# Autodesk Inventor assembly: Сборка ручка упрощённая
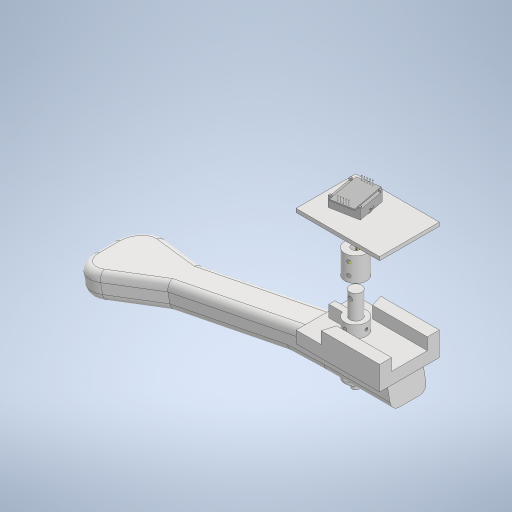
[picture p0: Inventor's stored thumbnail of the model, 512x512]
Saved by Autodesk Inventor 2023 (Build 270158000, 158)
## iProperties
Created: 2022-05-02
Part Number: Сборка ручка упрощённая
Document SubType Name: Assembly
Designer: User
Author: User
## Documents named in this file (10)
- C:\Users\avkap\Desktop\Стойка\Механизм ручки\Сборка ручка упрощённая.iam
- C:\Users\avkap\Desktop\Стойка\Механизм ручки\EAW.ipt
- C:\Users\avkap\Desktop\Стойка\Механизм ручки\Вал ручки.ipt
- C:\Users\avkap\Desktop\Стойка\Механизм ручки\Втулка энкодер.ipt
- C:\Users\avkap\Desktop\Стойка\Механизм ручки\Ручка.ipt
- C:\Users\avkap\Desktop\Стойка\Механизм ручки\Стенка.ipt
- C:\Users\avkap\Desktop\Стойка\Механизм ручки\Стопор.ipt
- C:\Users\avkap\Desktop\Стойка\Механизм ручки\Стенка энкодер.ipt
- C:\Users\avkap\Desktop\Стойка\Механизм ручки\М3х8.ipt
- C:\Users\avkap\Desktop\Стойка\Механизм ручки\Диск конец вала.ipt
## Components (9 placed, 9 different names)
1. EAW:1 — Цилиндрический:4
2. Вал ручки:1 — Цилиндрический:1, Совмещение:1, Цилиндрический:2, Цилиндрический:5, Совмещение:2, Цилиндрический:12
3. Втулка энкодер:1 — Цилиндрический:3, Цилиндрический:4
4. Ручка:1 — Цилиндрический:1, Совмещение:1
5. Стенка:1 — Заподлицо:1, Заподлицо:2, Цилиндрический:5, Совмещение:3
6. Стопор:1 — Цилиндрический:2, Совмещение:2, Совмещение:3
7. Стенка энкодер:1 — Заподлицо:1, Цилиндрический:3, Заподлицо:2
8. М3х8:1 — Цилиндрический:11, Цилиндрический:12
9. Диск конец вала:1 — Цилиндрический:11
## Relationships (12: CylindricalJoint 7, Mate 3, Flush 2)
- Цилиндрический:1 [CylindricalJoint]: Вал ручки:1 ↔ Ручка:1
- Совмещение:1 [Mate]: Вал ручки:1 ↔ Ручка:1
- Цилиндрический:2 [CylindricalJoint]: Вал ручки:1 ↔ Стопор:1
- Заподлицо:1 [Flush]: Стенка:1 ↔ Стенка энкодер:1
- Цилиндрический:3 [CylindricalJoint]: Втулка энкодер:1 ↔ Стенка энкодер:1
- Цилиндрический:4 [CylindricalJoint]: EAW:1 ↔ Втулка энкодер:1
- Заподлицо:2 [Flush]: Стенка:1 ↔ Стенка энкодер:1
- Цилиндрический:5 [CylindricalJoint]: Вал ручки:1 ↔ Стенка:1
- Совмещение:2 [Mate]: Вал ручки:1 ↔ Стопор:1
- Совмещение:3 [Mate]: Стенка:1 ↔ Стопор:1
- Цилиндрический:11 [CylindricalJoint]: М3х8:1 ↔ Диск конец вала:1
- Цилиндрический:12 [CylindricalJoint]: Вал ручки:1 ↔ М3х8:1
